# Autodesk Inventor assembly: strut_assem_UH
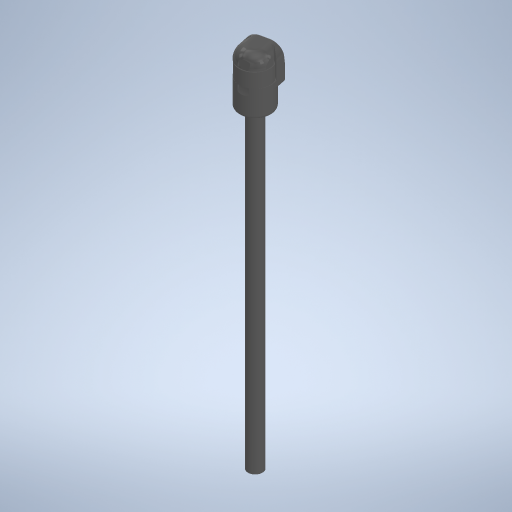
[picture p0: Inventor's stored thumbnail of the model, 512x512]
Saved by Autodesk Inventor 2024 (Build 280153000, 153)
## iProperties
Created: 2019-04-24
Part Number: strut_assem_UH
Document SubType Name: Assembly
Designer: Ishaan
Sending System: SolidWorks 2018
Last Author: Daniel Angeles
Last Saved: 2019-04-24
Author: Ishaan
## Documents named in this file (3)
- E:\Projects\Axiom--IDEX-3D-Printer\CAD\00 - COTS Components\Gas Strut Hardware\strut_assem\strut_assem_UH.iam
- E:\Projects\Axiom--IDEX-3D-Printer\CAD\00 - COTS Components\Gas Strut Hardware\strut_assem\end_mounts.ipt
- E:\Projects\Axiom--IDEX-3D-Printer\CAD\00 - COTS Components\Gas Strut Hardware\strut_assem\Part1^strut_assem.ipt
## Components (2 placed, 2 different names)
1. end_mounts:2 — Insert:1
2. Part1^strut_assem:1 — Insert:1
## Relationships (1: Insert 1)
- Insert:1: end_mounts:2 ↔ Part1^strut_assem:1
